# Autodesk Inventor assembly: CableBraider
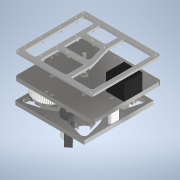
[picture p0: Inventor's stored thumbnail of the model, 180x180]
Saved by Autodesk Inventor 2022 (Build 260153070, 153G)
## iProperties
Created: 2020-07-21
Part Number: CableBraider
Document SubType Name: Assembly
Designer: elmar
Author: elmar
## Documents named in this file (13)
- D:\FourWireBraidingMachine\MetalCableBraider\CableBraider.iam
- D:\FourWireBraidingMachine\MetalCableBraider\BasePlate.ipt
- D:\FourWireBraidingMachine\MetalCableBraider\WinderAssembly.iam
- D:\FourWireBraidingMachine\MetalCableBraider\Carriage.iam
- D:\FourWireBraidingMachine\MetalCableBraider\NEMA17.ipt
- D:\FourWireBraidingMachine\MetalCableBraider\ElectronicsPlate.ipt
- D:\FourWireBraidingMachine\MetalCableBraider\DriveGearNEMA17.ipt
- D:\FourWireBraidingMachine\MetalCableBraider\TwoPartHornGear.ipt
- D:\FourWireBraidingMachine\MetalCableBraider\GuidePlate.ipt
- D:\FourWireBraidingMachine\MetalCableBraider\HornGearShaft.ipt
- C:\Users\elmar\OneDrive\Documents\Inventor\Content Center Files\R2022\en-US\DIN 934\DIN 934 - M8 x 1.25.ipt
- C:\Users\elmar\OneDrive\Documents\Inventor\Content Center Files\R2022\en-US\DIN 934\DIN 934 - M7 x 1.ipt
- D:\FourWireBraidingMachine\MetalCableBraider\Standoff.ipt
## Components (15 placed, 12 different names)
1. BasePlate:1 — Mate:1, Mate:2, Mate:3, Mate:10, Mate:13, Mate:14, Insert:1, Insert:2, Mate:16, Insert:4, Insert:6, Insert:7, Insert:8, Insert:9, Angle:10
2. TwoPartHornGear:1 — Angle:3, Flush:3, Insert:2, Flush:4
3. TwoPartHornGear:2 — Angle:3, Mate:16, Flush:4
4. WinderAssembly:1 [sub-assembly]
5. Carriage:1 [sub-assembly] — Mate:15, Tangent:1, Tangent:2
6. NEMA17:1 — Mate:10, Mate:12, Angle:4, Insert:1
7. ElectronicsPlate:1
8. DriveGearNEMA17:1 — Mate:12, Flush:3, Angle:4
9. GuidePlate:1 — Mate:13, Mate:14, Mate:15, Insert:3, Insert:5, Angle:8, Insert:10, Angle:9, Tangent:1, Tangent:2
10. HornGearShaft:1 — Insert:3, Angle:9
11. HornGearShaft:2 — Insert:4, Angle:10
12. DIN 934 - replaced by DIN EN 24032/28673/28674 M8:1 — Insert:5
13. DIN 934 - replaced by DIN EN 24032/28673/28674 M7:1 — Insert:6
14. DIN 934 - replaced by DIN EN 24032/28673/28674 M7:5 — Insert:7
15. Standoff:1 — Insert:8, Angle:8, Insert:9, Insert:10
## Relationships (28: Insert 10, Mate 9, Angle 5, Flush 2, Tangent 2)
- Mate:1: BasePlate:1
- Mate:2: BasePlate:1
- Mate:3: BasePlate:1
- Angle:3 (0 deg): TwoPartHornGear:1 ↔ TwoPartHornGear:2
- Mate:10: BasePlate:1 ↔ NEMA17:1
- Mate:12: NEMA17:1 ↔ DriveGearNEMA17:1
- Flush:3: TwoPartHornGear:1 ↔ DriveGearNEMA17:1
- Angle:4 (180 deg): NEMA17:1 ↔ DriveGearNEMA17:1
- Mate:13: BasePlate:1 ↔ GuidePlate:1
- Mate:14 (40 mm): BasePlate:1 ↔ GuidePlate:1
- Mate:15: Carriage:1 ↔ GuidePlate:1
- Insert:1: BasePlate:1 ↔ NEMA17:1
- Insert:2 (1.6 mm): BasePlate:1 ↔ TwoPartHornGear:1
- Mate:16: BasePlate:1 ↔ TwoPartHornGear:2
- Flush:4: TwoPartHornGear:1 ↔ TwoPartHornGear:2
- Insert:3: GuidePlate:1 ↔ HornGearShaft:1
- Insert:4: BasePlate:1 ↔ HornGearShaft:2
- Insert:5: GuidePlate:1 ↔ DIN 934 - replaced by DIN EN 24032/28673/28674 M8:1
- Insert:6: BasePlate:1 ↔ DIN 934 - replaced by DIN EN 24032/28673/28674 M7:1
- Insert:7: BasePlate:1 ↔ DIN 934 - replaced by DIN EN 24032/28673/28674 M7:5
- Insert:8: BasePlate:1 ↔ Standoff:1
- Angle:8 (0 deg): GuidePlate:1 ↔ Standoff:1
- Insert:9: BasePlate:1 ↔ Standoff:1
- Insert:10: GuidePlate:1 ↔ Standoff:1
- Angle:9 (0 deg): GuidePlate:1 ↔ HornGearShaft:1
- Angle:10 (0 deg): BasePlate:1 ↔ HornGearShaft:2
- Tangent:1: Carriage:1 ↔ GuidePlate:1
- Tangent:2: Carriage:1 ↔ GuidePlate:1
